# Autodesk Inventor assembly: LP_003
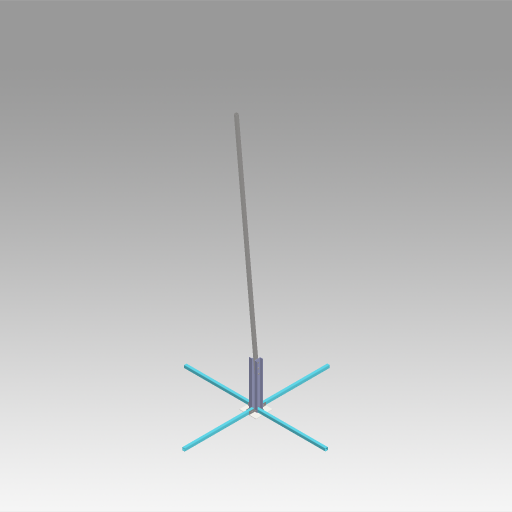
[picture p0: Inventor's stored thumbnail of the model, 512x512]
Saved by Autodesk Inventor 2023 (Build 270158000, 158)
## iProperties
Created: 2025-04-10
Part Number: LP_003
Document SubType Name: Assembly
Designer: NELLY NDUNG'U
Mass: 85996.3 g
Surface Area: 40567.1 cm^2
Volume: 10954.9 cm^3
Density: 7.85 g/cm^3
Author: NELLY NDUNG'U
## Documents named in this file (14)
- N:\NAKUJA\CAD FILES\AIRFRAME\LP003\LP_003.iam
- N:\NAKUJA\CAD FILES\AIRFRAME\LP003\BASE_ASSEMBLY.iam
- N:\NAKUJA\CAD FILES\AIRFRAME\LP003\RAIL_SUPPORT_50.iam
- C:\Users\User\Documents\Inventor\Content Center Files\R2023\en-US\ANSI B18.2.3.5M\ANSI B18.2.3.5M - M16 x 2 x 80.ipt
- C:\Users\User\Documents\Inventor\Content Center Files\R2023\en-US\ANSI B 18.2.4.1 M(1)\ANSI B 18.2.4.1 M - M16 x 2Style 1.ipt
- C:\Users\User\Documents\Inventor\Content Center Files\R2023\en-US\ANSI B18.2.3.5M\ANSI B18.2.3.5M - M16 x 2 x 75.ipt
- N:\NAKUJA\CAD FILES\AIRFRAME\LP003\LP_003\AIP\FEA\f138a9vuo.fins
- N:\NAKUJA\CAD FILES\AIRFRAME\LP003\LP_003\AIP\FEA\f138a9x0g.fsat
- N:\NAKUJA\CAD FILES\AIRFRAME\LP003\LP_003\AIP\FEA\f138a9xnk.ftes
- N:\NAKUJA\CAD FILES\AIRFRAME\LP003\LP_003\AIP\FEA\f138a9xnk.fwiz
- N:\NAKUJA\CAD FILES\AIRFRAME\LP003\LP_003\AIP\FEA\f138aa068.fmsh
- N:\NAKUJA\CAD FILES\AIRFRAME\LP003\LP_003\AIP\FEA\f138aa074.fres
- N:\NAKUJA\CAD FILES\AIRFRAME\LP003\LP_003\AIP\FEA\f15vwrd7k.fmsh
- N:\NAKUJA\CAD FILES\AIRFRAME\LP003\LP_003\AIP\FEA\f15vwrd7l.fres
## Components (12 placed, 5 different names)
1. BASE_ASSEMBLY:1 [sub-assembly] — Angle:1, Mate:1, Mate:2, Mate:3, Insert:1, Insert:2, Insert:3, Insert:4, Insert:5, Insert:6, Insert:7, Insert:8, Insert:9, Insert:10
2. RAIL_SUPPORT_50:1 [sub-assembly] — Angle:1, Mate:1, Mate:2, Mate:3
3. Hex Bolt - Metric M16 x 2 x 80:1 — Insert:1
4. Hex Bolt - Metric M16 x 2 x 80:2 — Insert:2
5. Hex Bolt - Metric M16 x 2 x 80:3 — Insert:3
6. Hex Nut Metric M16 x 2:1 — Insert:4
7. Hex Nut Metric M16 x 2:2 — Insert:5
8. Hex Nut Metric M16 x 2:3 — Insert:6
9. Hex Bolt - Metric M16 x 2 x 75:1 — Insert:7
10. Hex Bolt - Metric M16 x 2 x 75:2 — Insert:8
11. Hex Nut Metric M16 x 2:4 — Insert:9
12. Hex Nut Metric M16 x 2:5 — Insert:10
## Relationships (14: Insert 10, Mate 3, Angle 1)
- Angle:1 (85 deg): BASE_ASSEMBLY:1 ↔ RAIL_SUPPORT_50:1
- Mate:1 (-300 mm): BASE_ASSEMBLY:1 ↔ RAIL_SUPPORT_50:1
- Mate:2: BASE_ASSEMBLY:1 ↔ RAIL_SUPPORT_50:1
- Mate:3 (-5 mm): BASE_ASSEMBLY:1 ↔ RAIL_SUPPORT_50:1
- Insert:1: BASE_ASSEMBLY:1 ↔ Hex Bolt - Metric M16 x 2 x 80:1
- Insert:2: BASE_ASSEMBLY:1 ↔ Hex Bolt - Metric M16 x 2 x 80:2
- Insert:3: BASE_ASSEMBLY:1 ↔ Hex Bolt - Metric M16 x 2 x 80:3
- Insert:4: BASE_ASSEMBLY:1 ↔ Hex Nut Metric M16 x 2:1
- Insert:5: BASE_ASSEMBLY:1 ↔ Hex Nut Metric M16 x 2:2
- Insert:6: BASE_ASSEMBLY:1 ↔ Hex Nut Metric M16 x 2:3
- Insert:7: BASE_ASSEMBLY:1 ↔ Hex Bolt - Metric M16 x 2 x 75:1
- Insert:8: BASE_ASSEMBLY:1 ↔ Hex Bolt - Metric M16 x 2 x 75:2
- Insert:9: BASE_ASSEMBLY:1 ↔ Hex Nut Metric M16 x 2:4
- Insert:10: BASE_ASSEMBLY:1 ↔ Hex Nut Metric M16 x 2:5
## Named parameters: sa_0 = 412500, sa_1 = 412500
note: some values were not read from the file. Shown as the stored number, unit unknown: "sa_0", "sa_1".
